# Autodesk Inventor assembly: Ammonia Filter
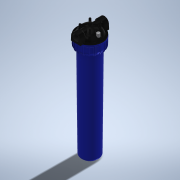
[picture p0: Inventor's stored thumbnail of the model, 180x180]
Saved by Autodesk Inventor 2020 (Build 240168000, 168)
## iProperties
Created: 2019-03-28
Part Number: Ammonia Filter
Material: Ogólny
Document SubType Name: Assembly
Designer: Marcin Kret
Mass: 1392.06 g
Surface Area: 4216.51 cm^2
Volume: 1062.64 cm^3
Density: 1.31 g/cm^3
Description: Filtr 10 mikronów
Vendor: AtlasFiltri
Author: Marcin Kret
## Documents named in this file (5)
- C:\Users\LENOVO\Desktop\Graduation Project\Fish Farming Unit\Water Loop Components\Ammonia Filter.iam
- C:\Users\LENOVO\Desktop\Graduation Project\Fish Farming Unit\Water Loop Components\master-plus-hot-3p-bfp-sx-ab-1.snapshot.2\Filtr HOT 3P -głowica.ipt
- C:\Users\LENOVO\Desktop\Graduation Project\Fish Farming Unit\Water Loop Components\master-plus-hot-3p-bfp-sx-ab-1.snapshot.2\Filtr HOT 3P -dzwon.ipt
- C:\Users\LENOVO\Desktop\Graduation Project\Fish Farming Unit\Water Loop Components\master-plus-hot-3p-bfp-sx-ab-1.snapshot.2\Filtr HOT 3P -nakrętka.ipt
- C:\Users\LENOVO\Desktop\Graduation Project\Fish Farming Unit\Water Loop Components\master-plus-hot-3p-bfp-sx-ab-1.snapshot.2\Filtr HOT 3P -korek.ipt
## Components (4 placed, 4 different names)
1. Filtr HOT 3P -głowica:1 — Sztywne:1, Sztywne:3
2. Filtr HOT 3P -dzwon:1 — Sztywne:1, Sztywne:2
3. Filtr HOT 3P -nakrętka:1 — Sztywne:2
4. Filtr HOT 3P -korek:1 — Sztywne:3
## Relationships (3: WeldJoint 3)
- Sztywne:1 [WeldJoint]: Filtr HOT 3P -głowica:1 ↔ Filtr HOT 3P -dzwon:1
- Sztywne:2 [WeldJoint]: Filtr HOT 3P -dzwon:1 ↔ Filtr HOT 3P -nakrętka:1
- Sztywne:3 [WeldJoint]: Filtr HOT 3P -głowica:1 ↔ Filtr HOT 3P -korek:1
